# Autodesk Inventor assembly: Wheel-Hub Assembly
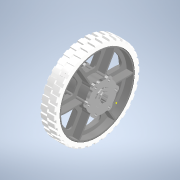
[picture p0: Inventor's stored thumbnail of the model, 180x180]
Saved by Autodesk Inventor 2020 (Build 240168000, 168)
## iProperties
Created: 2020-01-15
Part Number: Wheel-Hub Assembly
Document SubType Name: Assembly
Designer: 339294
Author: 339294
## Documents named in this file (3)
- \\prdshome32-33\home\33\339\339294\Desktop\2020\Wheels\Wheel-Hub Assembly.iam
- \\prdshome32-33\home\33\339\339294\Desktop\2020\Wheels\6in HiGrip WHeel.iam
- \\prdshome32-33\home\33\339\339294\Desktop\2020\Wheels\Hex Hub.ipt
## Components (3 placed, 2 different names)
1. 6in HiGrip WHeel:1 [sub-assembly] — Mate:1, Mate:2, Mate:4
2. Hex Hub:1 — Mate:1, Mate:2, Mate:3
3. Hex Hub:2 — Mate:3, Mate:4
## Relationships (4: Mate 4)
- Mate:1: 6in HiGrip WHeel:1 ↔ Hex Hub:1
- Mate:2: 6in HiGrip WHeel:1 ↔ Hex Hub:1
- Mate:3: Hex Hub:1 ↔ Hex Hub:2
- Mate:4: 6in HiGrip WHeel:1 ↔ Hex Hub:2
